# Autodesk Inventor assembly: inner
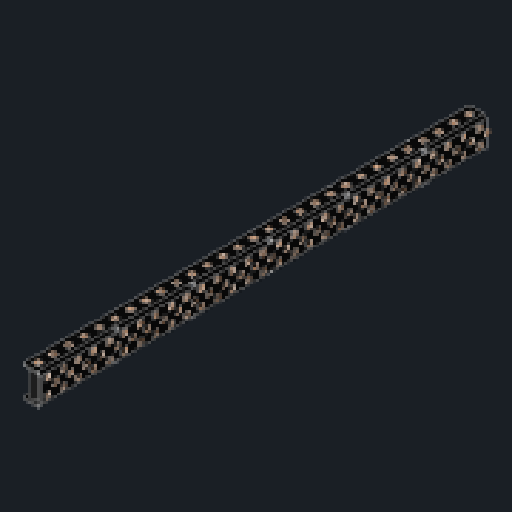
[picture p0: Inventor's stored thumbnail of the model, 512x512]
Saved by Autodesk Inventor 2024 (Build 280153000, 153)
## iProperties
Created: 2024-05-13
Part Number: inner
Document SubType Name: Assembly
Designer: Averey Ku
Author: Averey Ku
## Documents named in this file (5)
- D:\vex_robotics\hardware\cad\kdot\chassis\drivebay\inner.iam
- D:\vex_robotics\hardware\cad\VEX-CAD-Inventor-1.41\Structure\C Channel\Aluminum 1x2x1\Alu C 1x2x1x29.ipt
- D:\vex_robotics\hardware\cad\hardware\.375 OD Aluminum Spacer 0.875.ipt
- D:\vex_robotics\hardware\cad\VEX-CAD-Inventor-1.41\Electronics\Motors with Screws\SteelM-StarS.iam
- D:\vex_robotics\hardware\cad\VEX-CAD-Inventor-1.41\Electronics\Motors with Screws.iam
## Components (6 placed, 3 different names)
1. Alu C 1x2x1x29:1 — Insert:1, Insert:2, Insert:3, Mate:1, Insert:4, Insert:5, Mate:2
2. .375 OD Aluminum Spacer 0.875:1 — Insert:2
3. .375 OD Aluminum Spacer 0.875:2 — Insert:1
4. SteelM-StarS:1 [sub-assembly] — Insert:3, Mate:1
5. SteelM-StarS:2 [sub-assembly] — Insert:4
6. SteelM-StarS:3 [sub-assembly] — Insert:5, Mate:2
## Relationships (7: Insert 5, Mate 2)
- Insert:1: Alu C 1x2x1x29:1 ↔ .375 OD Aluminum Spacer 0.875:2
- Insert:2: Alu C 1x2x1x29:1 ↔ .375 OD Aluminum Spacer 0.875:1
- Insert:3: Alu C 1x2x1x29:1 ↔ SteelM-StarS:1
- Mate:1: Alu C 1x2x1x29:1 ↔ SteelM-StarS:1
- Insert:4: Alu C 1x2x1x29:1 ↔ SteelM-StarS:2
- Insert:5: Alu C 1x2x1x29:1 ↔ SteelM-StarS:3
- Mate:2: Alu C 1x2x1x29:1 ↔ SteelM-StarS:3
